# Autodesk Inventor assembly: case
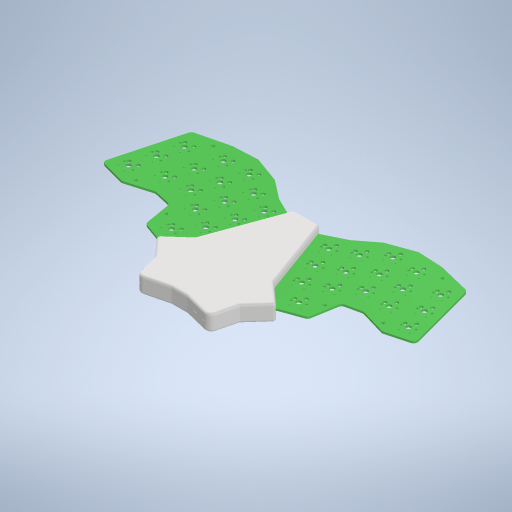
[picture p0: Inventor's stored thumbnail of the model, 512x512]
Saved by Autodesk Inventor 2024 (Build 280153000, 153)
## iProperties
Created: 2024-09-29
Part Number: case
Document SubType Name: Assembly
Designer: nikla
Author: nikla
## Documents named in this file (4)
- C:\Users\nikla\OneDrive\Keyboards\Blavinge\case\case.iam
- C:\Users\nikla\OneDrive\Keyboards\Blavinge\kicad\blavinge\blavinge.iam
- C:\Users\nikla\OneDrive\Keyboards\Blavinge\case\middle_top.ipt
- C:\Users\nikla\Desktop\middle_bottom.ipt
## Components (3 placed, 3 different names)
1. blavinge:1 [sub-assembly] — Fluchtend:1, Fluchtend:2
2. middle_top:1 — Fluchtend:1
3. middle_bottom:1 — Fluchtend:2
## Relationships (2: Flush 2)
- Fluchtend:1 [Flush]: blavinge:1 ↔ middle_top:1
- Fluchtend:2 [Flush]: blavinge:1 ↔ middle_bottom:1
